# Autodesk Inventor assembly: cover
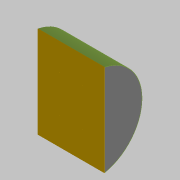
[picture p0: Inventor's stored thumbnail of the model, 180x180]
Saved by Autodesk Inventor 2021 (Build 250183000, 183)
## iProperties
Created: 2021-05-06
Part Number: cover
Document SubType Name: Assembly
Designer: Watchdog
Author: Watchdog
## Documents named in this file (5)
- C:\Users\Watchdog\OneDrive - Flinders\Advn Mech Design Shared\6_Development\2_Design\inventor\cover\cover.iam
- C:\Users\Watchdog\OneDrive - Flinders\Advn Mech Design Shared\6_Development\2_Design\inventor\cover\cover_base.ipt
- C:\Users\Watchdog\OneDrive - Flinders\Advn Mech Design Shared\6_Development\2_Design\inventor\cover\cover_shell.ipt
- C:\Users\Watchdog\OneDrive - Flinders\Advn Mech Design Shared\6_Development\2_Design\inventor\cover\cover_side.ipt
- C:\Users\Watchdog\OneDrive - Flinders\Advn Mech Design Shared\6_Development\2_Design\inventor\cover\cover_side_open.ipt
## Components (4 placed, 4 different names)
1. cover_base:1 — Mate:1, Mate:2, Mate:3, Mate:4, Mate:6, Mate:7, Mate:8, Mate:10, Mate:11, Flush:1, Flush:2, Symmetry:1
2. cover_shell:1 — Mate:3, Mate:4, Mate:9, Mate:12
3. cover_side:1 — Mate:7, Mate:8, Mate:9
4. cover_side_open:1 — Mate:10, Mate:11, Mate:12, Flush:1
## Relationships (14: Mate 11, Flush 2, Symmetry 1)
- Mate:1: cover_base:1
- Mate:2: cover_base:1
- Mate:3: cover_base:1 ↔ cover_shell:1
- Mate:4: cover_base:1 ↔ cover_shell:1
- Mate:6: cover_base:1
- Mate:7: cover_base:1 ↔ cover_side:1
- Mate:8: cover_base:1 ↔ cover_side:1
- Mate:9: cover_shell:1 ↔ cover_side:1
- Mate:10: cover_base:1 ↔ cover_side_open:1
- Mate:11: cover_base:1 ↔ cover_side_open:1
- Mate:12: cover_shell:1 ↔ cover_side_open:1
- Flush:1: cover_base:1 ↔ cover_side_open:1
- Flush:2: cover_base:1
- Symmetry:1: cover_base:1
